# Autodesk Inventor assembly: tensioner
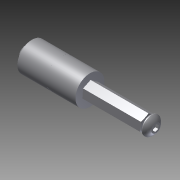
[picture p0: Inventor's stored thumbnail of the model, 180x180]
Saved by Autodesk Inventor 2014 SP1 (Build 180222100, 222)
## iProperties
Created: 2013-08-29
Part Number: tensioner
Document SubType Name: Assembly
Designer: Ryan
Sending System: SolidWorks 2013
Last Author: Ryan
Author: Ryan
## Documents named in this file (4)
- C:\Users\Ryan\Desktop\sw\toss up 4th robot\drive\tensioner.iam
- C:\Users\Ryan\Desktop\sw\lib\Aperture VEX CAD Library\Spacers\SPACER-0500-0500.ipt
- C:\Users\Ryan\Desktop\sw\lib\Aperture VEX CAD Library\Standoffs\BEAM-2000.ipt
- C:\Users\Ryan\Desktop\sw\lib\Aperture VEX CAD Library\Hardware\8-32\8-32_.375.ipt
## Components (5 placed, 4 different names)
1. spacer-0500-0500:1 — Mate:1, Mate:2, Mate:3, Flush:1, Mate:4, Mate:5
2. SPACER-0500-0500:2 — Mate:1, Mate:2
3. BEAM-2000:1 — Mate:3, Flush:1, Mate:6, Mate:7
4. 8-32_.375:1 — Mate:4, Mate:5
5. 8-32_.375:2 — Mate:6, Mate:7
## Relationships (8: Mate 7, Flush 1)
- Mate:1: spacer-0500-0500:1 ↔ SPACER-0500-0500:2
- Mate:2: spacer-0500-0500:1 ↔ SPACER-0500-0500:2
- Mate:3: spacer-0500-0500:1 ↔ BEAM-2000:1
- Flush:1: spacer-0500-0500:1 ↔ BEAM-2000:1
- Mate:4: spacer-0500-0500:1 ↔ 8-32_.375:1
- Mate:5 (1.1684 mm): spacer-0500-0500:1 ↔ 8-32_.375:1
- Mate:6: BEAM-2000:1 ↔ 8-32_.375:2
- Mate:7 (1.1684 mm): BEAM-2000:1 ↔ 8-32_.375:2
